# Autodesk Inventor assembly: Chuck Assembly
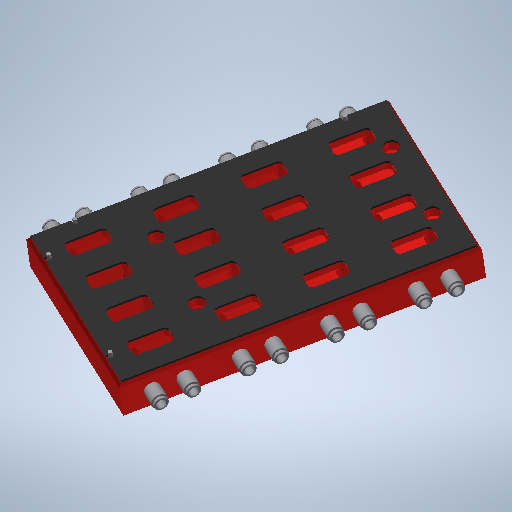
[picture p0: Inventor's stored thumbnail of the model, 512x512]
Saved by Autodesk Inventor 2025 (Build 290162000, 162)
## iProperties
Created: 2021-01-11
Part Number: Chuck Assembly
Document SubType Name: Assembly
Designer: caleb
Author: caleb
## Documents named in this file (6)
- C:\Users\cfang\Desktop\nebraska-silicon-lab\Hardware\ETL\Module Assembly\Chuck - 16-pocket V2\Chuck - 16-pocket - V2.iam
- C:\Users\cfang\Desktop\nebraska-silicon-lab\Hardware\ETL\Module Assembly\Chuck - 16-pocket V2\Chuck - 16-pocket - V2.ipt
- C:\Users\cfang\Desktop\nebraska-silicon-lab\Hardware\ETL\Module Assembly\Chuck - V3\93600A304_316 Stainless Steel Dowel Pin\93600A304_316 Stainless Steel Dowel Pin.ipt
- C:\Users\cfang\Desktop\nebraska-silicon-lab\Hardware\ETL\Module Assembly\BBM Staging Plate - V2\BBM Staging Plate Assembly - V2.iam
- C:\Users\cfang\Desktop\nebraska-silicon-lab\Hardware\ETL\Module Assembly\Chuck - 16-pocket V2\5111K573_Push-to-Connect Tube Fitting for Air and Water\5111K573_Push-to-Connect Tube Fitting for Air and Water.ipt
- C:\Users\cfang\Desktop\nebraska-silicon-lab\Hardware\ETL\Module Assembly\Chuck - 16-pocket V2\gasket V1.ipt
## Components (23 placed, 5 different names)
1. Chuck - 16-pocket - V2:1 — Insert:1, Insert:2, Insert:3, Insert:4, Mate:1, Angle:1, Insert:5, Insert:6, Insert:7, Insert:8, Insert:9, Insert:10, Insert:11, Insert:12, Insert:13, Insert:14, Insert:15, Insert:16, Insert:17, Insert:18, Insert:19, Insert:20, Mate:2, Insert:21, Insert:22
2. 93600A304_316 Stainless Steel Dowel Pin:1 — Insert:1, Tangent:2
3. 93600A304_316 Stainless Steel Dowel Pin:2 — Insert:2, Tangent:3
4. 93600A304_316 Stainless Steel Dowel Pin:3 — Insert:3, Tangent:1
5. 93600A304_316 Stainless Steel Dowel Pin:4 — Insert:4
6. BBM Staging Plate Assembly - V2:1 [sub-assembly] — Mate:1, Tangent:1, Tangent:2, Tangent:3, Angle:1
7. 5111K573_Push-to-Connect Tube Fitting for Air and Water:1 — Insert:5
8. 5111K573_Push-to-Connect Tube Fitting for Air and Water:2 — Insert:6
9. 5111K573_Push-to-Connect Tube Fitting for Air and Water:3 — Insert:7
10. 5111K573_Push-to-Connect Tube Fitting for Air and Water:4 — Insert:8
11. 5111K573_Push-to-Connect Tube Fitting for Air and Water:5 — Insert:10
12. 5111K573_Push-to-Connect Tube Fitting for Air and Water:6 — Insert:11
13. 5111K573_Push-to-Connect Tube Fitting for Air and Water:7 — Insert:9
14. 5111K573_Push-to-Connect Tube Fitting for Air and Water:8 — Insert:12
15. 5111K573_Push-to-Connect Tube Fitting for Air and Water:9 — Insert:13
16. 5111K573_Push-to-Connect Tube Fitting for Air and Water:10 — Insert:14
17. 5111K573_Push-to-Connect Tube Fitting for Air and Water:11 — Insert:15
18. 5111K573_Push-to-Connect Tube Fitting for Air and Water:12 — Insert:16
19. 5111K573_Push-to-Connect Tube Fitting for Air and Water:13 — Insert:17
20. 5111K573_Push-to-Connect Tube Fitting for Air and Water:14 — Insert:18
21. 5111K573_Push-to-Connect Tube Fitting for Air and Water:15 — Insert:19
22. 5111K573_Push-to-Connect Tube Fitting for Air and Water:16 — Insert:20
23. gasket V1:1 — Mate:2, Insert:21, Insert:22
## Relationships (28: Insert 22, Tangent 3, Mate 2, Angle 1)
- Insert:1 (-5 mm): Chuck - 16-pocket - V2:1 ↔ 93600A304_316 Stainless Steel Dowel Pin:1
- Insert:2 (-5 mm): Chuck - 16-pocket - V2:1 ↔ 93600A304_316 Stainless Steel Dowel Pin:2
- Insert:3 (-5 mm): Chuck - 16-pocket - V2:1 ↔ 93600A304_316 Stainless Steel Dowel Pin:3
- Insert:4 (-5 mm): Chuck - 16-pocket - V2:1 ↔ 93600A304_316 Stainless Steel Dowel Pin:4
- Mate:1: Chuck - 16-pocket - V2:1 ↔ BBM Staging Plate Assembly - V2:1
- Tangent:1: 93600A304_316 Stainless Steel Dowel Pin:3 ↔ BBM Staging Plate Assembly - V2:1
- Tangent:2: 93600A304_316 Stainless Steel Dowel Pin:1 ↔ BBM Staging Plate Assembly - V2:1
- Tangent:3: 93600A304_316 Stainless Steel Dowel Pin:2 ↔ BBM Staging Plate Assembly - V2:1
- Angle:1 (0 deg): Chuck - 16-pocket - V2:1 ↔ BBM Staging Plate Assembly - V2:1
- Insert:5: Chuck - 16-pocket - V2:1 ↔ 5111K573_Push-to-Connect Tube Fitting for Air and Water:1
- Insert:6: Chuck - 16-pocket - V2:1 ↔ 5111K573_Push-to-Connect Tube Fitting for Air and Water:2
- Insert:7: Chuck - 16-pocket - V2:1 ↔ 5111K573_Push-to-Connect Tube Fitting for Air and Water:3
- Insert:8: Chuck - 16-pocket - V2:1 ↔ 5111K573_Push-to-Connect Tube Fitting for Air and Water:4
- Insert:9: Chuck - 16-pocket - V2:1 ↔ 5111K573_Push-to-Connect Tube Fitting for Air and Water:7
- Insert:10: Chuck - 16-pocket - V2:1 ↔ 5111K573_Push-to-Connect Tube Fitting for Air and Water:5
- Insert:11: Chuck - 16-pocket - V2:1 ↔ 5111K573_Push-to-Connect Tube Fitting for Air and Water:6
- Insert:12: Chuck - 16-pocket - V2:1 ↔ 5111K573_Push-to-Connect Tube Fitting for Air and Water:8
- Insert:13: Chuck - 16-pocket - V2:1 ↔ 5111K573_Push-to-Connect Tube Fitting for Air and Water:9
- Insert:14: Chuck - 16-pocket - V2:1 ↔ 5111K573_Push-to-Connect Tube Fitting for Air and Water:10
- Insert:15: Chuck - 16-pocket - V2:1 ↔ 5111K573_Push-to-Connect Tube Fitting for Air and Water:11
- Insert:16: Chuck - 16-pocket - V2:1 ↔ 5111K573_Push-to-Connect Tube Fitting for Air and Water:12
- Insert:17: Chuck - 16-pocket - V2:1 ↔ 5111K573_Push-to-Connect Tube Fitting for Air and Water:13
- Insert:18: Chuck - 16-pocket - V2:1 ↔ 5111K573_Push-to-Connect Tube Fitting for Air and Water:14
- Insert:19: Chuck - 16-pocket - V2:1 ↔ 5111K573_Push-to-Connect Tube Fitting for Air and Water:15
- Insert:20: Chuck - 16-pocket - V2:1 ↔ 5111K573_Push-to-Connect Tube Fitting for Air and Water:16
- Mate:2: Chuck - 16-pocket - V2:1 ↔ gasket V1:1
- Insert:21: Chuck - 16-pocket - V2:1 ↔ gasket V1:1
- Insert:22: Chuck - 16-pocket - V2:1 ↔ gasket V1:1
